# Autodesk Inventor assembly: Bumper v2
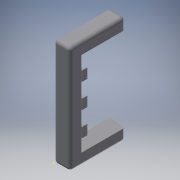
[picture p0: Inventor's stored thumbnail of the model, 180x180]
Saved by Autodesk Inventor 2018 (Build 220112000, 112)
## iProperties
Created: 2018-09-24
Part Number: Bumper v2
Document SubType Name: Assembly
Designer: maste
Author: maste
## Documents named in this file (4)
- C:\Users\maste\Desktop\Summer Drive Base V1\Summer Drivebase\Bumper v2.iam
- C:\Users\maste\Desktop\Summer Drive Base V1\Summer Drivebase\Bumper v2.ipt
- C:\Users\maste\Desktop\Summer Drive Base V1\Summer Drivebase\Beefy L.ipt
- C:\Users\maste\Desktop\Summer Drive Base V1\Summer Drivebase\Beefy Spacer.ipt
## Components (7 placed, 3 different names)
1. Bumper v2:1 — Mate:10, Mate:11, Mate:12, Mate:13, Mate:14, Mate:15, Mate:16, Mate:17, Mate:18
2. Beefy L:1 — Mate:7, Mate:8, Mate:9
3. Beefy L:2 — Mate:4, Mate:5, Mate:6
4. Beefy L:3 — Mate:1, Mate:2, Mate:3
5. Beefy Spacer:1 — Mate:1, Mate:2, Mate:3, Mate:13, Mate:14, Mate:15
6. Beefy Spacer:2 — Mate:4, Mate:5, Mate:6, Mate:10, Mate:11, Mate:12
7. Beefy Spacer:3 — Mate:7, Mate:8, Mate:9, Mate:16, Mate:17, Mate:18
## Relationships (18: Mate 18)
- Mate:1: Beefy L:3 ↔ Beefy Spacer:1
- Mate:2: Beefy L:3 ↔ Beefy Spacer:1
- Mate:3: Beefy L:3 ↔ Beefy Spacer:1
- Mate:4: Beefy L:2 ↔ Beefy Spacer:2
- Mate:5: Beefy L:2 ↔ Beefy Spacer:2
- Mate:6: Beefy L:2 ↔ Beefy Spacer:2
- Mate:7: Beefy L:1 ↔ Beefy Spacer:3
- Mate:8: Beefy L:1 ↔ Beefy Spacer:3
- Mate:9: Beefy L:1 ↔ Beefy Spacer:3
- Mate:10: Bumper v2:1 ↔ Beefy Spacer:2
- Mate:11: Bumper v2:1 ↔ Beefy Spacer:2
- Mate:12: Bumper v2:1 ↔ Beefy Spacer:2
- Mate:13: Bumper v2:1 ↔ Beefy Spacer:1
- Mate:14: Bumper v2:1 ↔ Beefy Spacer:1
- Mate:15: Bumper v2:1 ↔ Beefy Spacer:1
- Mate:16: Bumper v2:1 ↔ Beefy Spacer:3
- Mate:17: Bumper v2:1 ↔ Beefy Spacer:3
- Mate:18: Bumper v2:1 ↔ Beefy Spacer:3
